# Autodesk Inventor assembly: ManganPitik
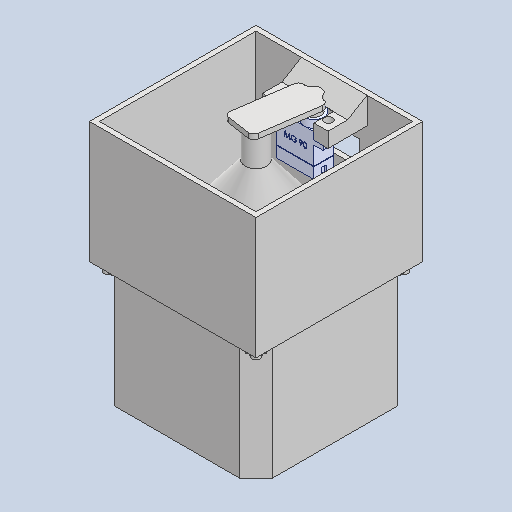
[picture p0: Inventor's stored thumbnail of the model, 512x512]
Saved by Autodesk Inventor 2026.2 (Build 302298010, 298A)
## iProperties
Created: 2026-05-22
Part Number: ManganPitik
Document SubType Name: Assembly
Designer: rizky
Author: rizky
## Documents named in this file (5)
- C:\SEMESTER 4\Mikrokontroller\PakanPitik\ManganPitik.iam
- C:\SEMESTER 4\TEKNOFEST\Robolig\GripperGeser\servo-motor-sg90-mg90-1.snapshot.9\mg 90 micro servo\mg 90 micro servo\mg 90 micro servo.ipt
- C:\SEMESTER 4\Mikrokontroller\PakanPitik\TutupTank.ipt
- C:\SEMESTER 4\Mikrokontroller\PakanPitik\CorongBawah.ipt
- C:\SEMESTER 4\Mikrokontroller\PakanPitik\Tank.ipt
## Components (4 placed, 4 different names)
1. mg 90 micro servo:1 — Mate:5, Mate:6, Mate:7, Mate:8, Mate:9
2. CorongBawah:1 — Mate:5, Mate:8, Mate:9, Mate:10, Mate:11, Mate:12
3. TutupTank:1 — Mate:6, Mate:7
4. Tank:1 — Mate:10, Mate:11, Mate:12
## Relationships (8: Mate 8)
- Mate:5: mg 90 micro servo:1 ↔ CorongBawah:1
- Mate:6: mg 90 micro servo:1 ↔ TutupTank:1
- Mate:7: mg 90 micro servo:1 ↔ TutupTank:1
- Mate:8: mg 90 micro servo:1 ↔ CorongBawah:1
- Mate:9: mg 90 micro servo:1 ↔ CorongBawah:1
- Mate:10: CorongBawah:1 ↔ Tank:1
- Mate:11: CorongBawah:1 ↔ Tank:1
- Mate:12: CorongBawah:1 ↔ Tank:1
